# Autodesk Inventor assembly: Tilted Camera Assembly
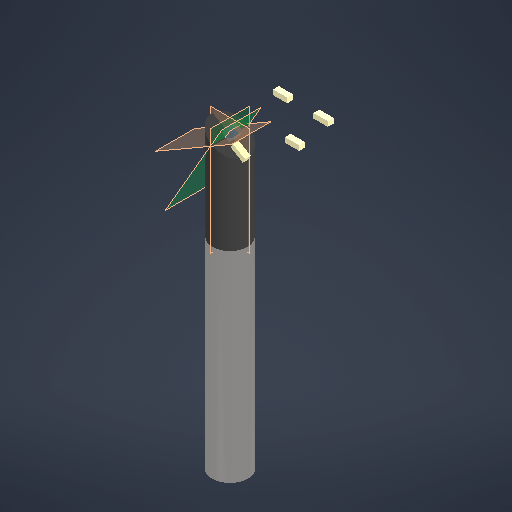
[picture p0: Inventor's stored thumbnail of the model, 512x512]
Saved by Autodesk Inventor 2026.2 (Build 302298010, 298A)
## iProperties
Created: 2026-04-01
Part Number: Tilted Camera Assembly
Document SubType Name: Assembly
Designer: piete
Author: piete
## Documents named in this file (5)
- C:\Users\piete\Desktop\Skripsie\Documents\Concept Designs\Concept 2 Tilted Camera design\Tilted Camera Assembly.iam
- C:\Users\piete\Desktop\Skripsie\Documents\Concept Designs\Concept 2 Tilted Camera design\Shaft.ipt
- C:\Users\piete\Desktop\Skripsie\Documents\Concept Designs\Concept 2 Tilted Camera design\Camera encasing.ipt
- C:\Users\piete\Desktop\Skripsie\Documents\Concept Designs\Camera sensor.ipt
- C:\Users\piete\Desktop\Skripsie\Documents\Concept Designs\Large light.ipt
## Components (7 placed, 4 different names)
1. Shaft:1 — Mate:1, Mate:2, Flush:1
2. Camera encasing:1 — Mate:1, Mate:2, Flush:1, Mate:3, Flush:2, Flush:3, Mate:4
3. Camera sensor:1 — Mate:3, Flush:2, Flush:3
4. Large light:1
5. Large light:2
6. Large light:3 — Mate:4
7. Large light:4
## Relationships (7: Mate 4, Flush 3)
- Mate:1: Shaft:1 ↔ Camera encasing:1
- Mate:2: Shaft:1 ↔ Camera encasing:1
- Flush:1: Shaft:1 ↔ Camera encasing:1
- Mate:3: Camera encasing:1 ↔ Camera sensor:1
- Flush:2 (-1 mm): Camera encasing:1 ↔ Camera sensor:1
- Flush:3: Camera encasing:1 ↔ Camera sensor:1
- Mate:4: Camera encasing:1 ↔ Large light:3
